# Autodesk Inventor assembly: Actuator
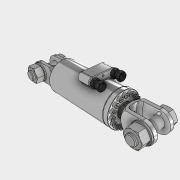
[picture p0: Inventor's stored thumbnail of the model, 180x180]
Saved by Autodesk Inventor 2020.1 (Build 241239000, 239)
## iProperties
Created: 2019-09-17
Part Number: Actuator
Document SubType Name: Assembly
Designer: thomastremblay
Author: thomastremblay
## Documents named in this file (3)
- C:\Users\thom_tremblay\Desktop\Inventor ACP Data\Actuator.iam
- C:\Users\thom_tremblay\Desktop\Inventor ACP Data\Assemblies\Piston_Housing.iam
- C:\Users\thom_tremblay\Desktop\Inventor ACP Data\Assemblies\Piston_Rod.iam
## Components (2 placed, 2 different names)
1. Piston_Housing:1 [sub-assembly] — Actuator Stroke
2. Piston_Rod:1 [sub-assembly] — Actuator Stroke
## Relationships (3: Mate 2, Angle 1)
- [Mate]: Piston_Housing:1 ↔ Piston_Rod:1
- [Angle] (0 deg): Piston_Housing:1 ↔ Piston_Rod:1
- Actuator Stroke [Mate]: Piston_Housing:1 ↔ Piston_Rod:1
